# Autodesk Inventor assembly: 2020RobotV05
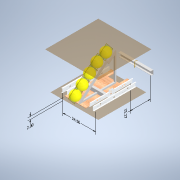
[picture p0: Inventor's stored thumbnail of the model, 180x180]
Saved by Autodesk Inventor 2020.2 (Build 242310000, 310)
## iProperties
Created: 2020-01-12
Part Number: 2020RobotV05
Document SubType Name: Assembly
Designer: robst
Author: robst
## Documents named in this file (17)
- C:\git\CAD-Development\robSteele\2020LongRobotBase\2020RobotV05.iam
- C:\git\CAD-Development\robSteele\2020LongRobotBase\2020 End Plate.ipt
- C:\git\CAD-Development\robSteele\2020LongRobotBase\am-3921 AM14U4 Outside Plate.ipt
- C:\git\CAD-Development\robSteele\2020LongRobotBase\am-3922 AM14U4 Inside Plate.ipt
- C:\git\CAD-Development\robSteele\2020LongRobotBase\crossPlate.ipt
- C:\git\CAD-Development\robSteele\2020LongRobotBase\floor.ipt
- C:\git\CAD-Development\robSteele\2020LongRobotBase\1892-YEL.ipt
- C:\git\CAD-Development\robSteele\2020LongRobotBase\ceiling.ipt
- C:\git\CAD-Development\robSteele\2020LiftMechanism\primativeBaseForShortRobot.ipt
- C:\git\CAD-Development\robSteele\2020LiftMechanism\primative1stStageForShortRobot.ipt
- C:\git\CAD-Development\robSteele\2020LiftMechanism\primative4thStageForShortRobot.ipt
- C:\git\CAD-Development\robSteele\2020LiftMechanism\primative3rdStageForShortRobot.ipt
- C:\git\CAD-Development\robSteele\2020LongRobotBase\ballRampLeftSideV04.ipt
- C:\git\CAD-Development\robSteele\2020LongRobotBase\2020 Wood BaseV04.ipt
- C:\git\CAD-Development\robSteele\2020LongRobotBase\ballRampRightSideV04.ipt
- C:\git\CAD-Development\robSteele\2020LongRobotBase\ballRampWithPocketForPowerCell.ipt
- C:\git\CAD-Development\robSteele\2020LongRobotBase\ballRampWithPocketForPowerCell_MIR.ipt
## Components (22 placed, 16 different names)
1. 2020 End Plate:1
2. am-3921 AM14U4 Outside Plate:1 — Mate:15
3. am-3921 AM14U4 Outside Plate:2 — Mate:9
4. am-3922 AM14U4 Inside Plate:1 — Mate:9, Mate:12, Flush:4, Flush:5
5. crossPlate:1 — Mate:12, Flush:4, Flush:5
6. am-3922 AM14U4 Inside Plate:2 — Mate:15
7. floor:1 — Mate:54, Mate:55, Flush:18, Mate:65
8. 1892-YEL:1 — Mate:83, Mate:88
9. 1892-YEL:2 — Mate:84, Mate:89
10. 1892-YEL:3 — Mate:86, Mate:91
11. 1892-YEL:4 — Mate:85, Mate:90
12. 1892-YEL:5 — Mate:79, Mate:87, Mate:92
13. ceiling:1 — Mate:65
14. 2020 Wood BaseV04:1 — Mate:54, Mate:93, Mate:94
15. primativeBaseForShortRobot:1 — Mate:40
16. primative1stStageForShortRobot:1 — Mate:40, Mate:43
17. primative3rdStageForShortRobot:1 — Mate:43, Mate:45
18. primative4thStageForShortRobot:1 — Mate:45
19. ballRampLeftSideV04:1 — Mate:70
20. ballRampRightSideV04:1
21. ballRampWithPocketForPowerCell:1 — Mate:82, Mate:83, Mate:84, Mate:85, Mate:86, Mate:87
22. ballRampWithPocketForPowerCell_MIR:1 — Flush:31
## Relationships (28: Mate 24, Flush 4)
- Mate:9 (85.725 mm): am-3921 AM14U4 Outside Plate:2 ↔ am-3922 AM14U4 Inside Plate:1
- Mate:12: am-3922 AM14U4 Inside Plate:1 ↔ crossPlate:1
- Flush:4: am-3922 AM14U4 Inside Plate:1 ↔ crossPlate:1
- Flush:5 (304.8 mm): am-3922 AM14U4 Inside Plate:1 ↔ crossPlate:1
- Mate:15 (85.725 mm): am-3921 AM14U4 Outside Plate:1 ↔ am-3922 AM14U4 Inside Plate:2
- Mate:40 (12.7 mm): primativeBaseForShortRobot:1 ↔ primative1stStageForShortRobot:1
- Mate:43 (12.7 mm): primative1stStageForShortRobot:1 ↔ primative3rdStageForShortRobot:1
- Mate:45 (12.7 mm): primative3rdStageForShortRobot:1 ↔ primative4thStageForShortRobot:1
- Mate:54 (50.8 mm): floor:1 ↔ 2020 Wood BaseV04:1
- Mate:55: floor:1
- Flush:18: floor:1
- Mate:65 (711.2 mm): floor:1 ↔ ceiling:1
- Mate:70 (57.15 mm): ballRampLeftSideV04:1
- Mate:79: 1892-YEL:5
- Mate:82 (57.15 mm): ballRampWithPocketForPowerCell:1
- Flush:31 (-57.15 mm): ballRampWithPocketForPowerCell_MIR:1
- Mate:83: 1892-YEL:1 ↔ ballRampWithPocketForPowerCell:1
- Mate:84: 1892-YEL:2 ↔ ballRampWithPocketForPowerCell:1
- Mate:85: 1892-YEL:4 ↔ ballRampWithPocketForPowerCell:1
- Mate:86: 1892-YEL:3 ↔ ballRampWithPocketForPowerCell:1
- Mate:87: 1892-YEL:5 ↔ ballRampWithPocketForPowerCell:1
- Mate:88: 1892-YEL:1
- Mate:89: 1892-YEL:2
- Mate:90: 1892-YEL:4
- Mate:91: 1892-YEL:3
- Mate:92: 1892-YEL:5
- Mate:93: 2020 Wood BaseV04:1
- Mate:94: 2020 Wood BaseV04:1
## Named parameters: centerLineToEdgeOffBallRamp = 57.15 mm
